# Autodesk Inventor assembly: PBD-14
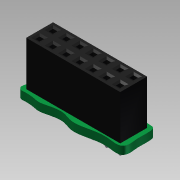
[picture p0: Inventor's stored thumbnail of the model, 180x180]
Saved by Autodesk Inventor 2011 (Build 150239000, 239)
## iProperties
Created: 2011-01-23
Part Number: PBD-14
Document SubType Name: Assembly
Designer: Aleirim
Author: Aleirim
## Documents named in this file (3)
- D:\Abbath\Work\11.2\Сумматор light\КД\RSXX к сумматору\Установка элементов\PBD-14 установка.iam
- D:\Abbath\Work\11.2\Сумматор light\КД\RSXX к сумматору\Установка элементов\PBD-14.ipt
- D:\Abbath\Work\11.2\Сумматор light\КД\RSXX к сумматору\Установка элементов\PBD-14 плата.ipt
## Components (2 placed, 2 different names)
1. PBD-14:1 — Заподлицо:1
2. PBD-14 плата:1 — Заподлицо:1
## Relationships (1: Flush 1)
- Заподлицо:1 [Flush]: PBD-14:1 ↔ PBD-14 плата:1
